# Autodesk Inventor assembly: Gearbox
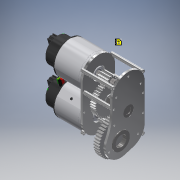
[picture p0: Inventor's stored thumbnail of the model, 180x180]
Saved by Autodesk Inventor 2019.4 (Build 234330000, 330)
## iProperties
Created: 2019-12-11
Part Number: Gearbox
Document SubType Name: Assembly
Designer: admin
Author: admin
## Documents named in this file (11)
- C:\Users\admin\Desktop\FRC 2020 Engineering\GitHub\Gearbox.iam
- C:\Users\admin\Desktop\FRC 2020 Engineering\GitHub\7738-CAD-prep\Swerve Module\Falcon_500_Powered_by_Talon_FX_217-6515.iam
- C:\Users\admin\Desktop\FRC 2020 Engineering\GitHub\7738-CAD-prep\WCD\10T_Steel_Spur_Gear_20_DP_12T_Center_Distance_Falcon_Motor_217-6917.ipt
- C:\Users\admin\Desktop\FRC 2020 Engineering\GitHub\40t_Aluminum_Spur_Gear_20_DP_1_2_Hex_Bore_217-2708.ipt
- C:\Users\admin\Desktop\FRC 2020 Engineering\GitHub\Gearbox\Design Accelerator\Spur Gears1.iam
- C:\Users\admin\Desktop\FRC 2020 Engineering\GitHub\7738-CAD-prep\Butterfly Drive Mk2\Butterfly Base\F6800Z 10mm ID Flange.ipt
- C:\Users\admin\Desktop\FRC 2020 Engineering\GitHub\Gearbox Plate 1.ipt
- C:\Users\admin\Desktop\FRC 2020 Engineering\GitHub\7738-CAD-prep\Butterfly Drive Mk2\Butterfly Module\F6004.ipt
- C:\Users\admin\Desktop\FRC 2020 Engineering\GitHub\Gearbox Plate 2.ipt
- C:\Users\admin\Desktop\FRC 2020 Engineering\GitHub\Shaft Jr.ipt
- C:\Users\admin\Desktop\FRC 2020 Engineering\GitHub\Spacer.ipt
## Components (18 placed, 10 different names)
1. Falcon_500_Powered_by_Talon_FX_217-6515:1 [sub-assembly] — Mate:2, Flush:1, Mate:5, Mate:7, Flush:4, Mate:11, Mate:15
2. Falcon_500_Powered_by_Talon_FX_217-6515:2 [sub-assembly] — Flush:1, Mate:3, Mate:4, Mate:6, Mate:9, Mate:13, Mate:14
3. 10T_Steel_Spur_Gear_20_DP_12T_Center_Distance_Falcon_Motor_217-6917:2 — Mate:2, Flush:2
4. 10T_Steel_Spur_Gear_20_DP_12T_Center_Distance_Falcon_Motor_217-6917:3 — Mate:3, Flush:2, Flush:3, Mate:9
5. 40t_Aluminum_Spur_Gear_20_DP_1_2_Hex_Bore_217-2708:1 — Flush:3, Mate:6, Mate:7, Mate:8, Mate:10
6. Spur Gears:1 [sub-assembly] — Mate:10, Mate:11, Mate:18, Mate:19, Mate:20
7. F6800Z 10mm ID Flange:1 — Mate:16, Mate:17, Mate:26
8. Gearbox Plate 1:1 — Mate:13, Mate:14, Mate:15, Mate:16, Mate:17
9. F6004:1 — Mate:21, Mate:22
10. Gearbox Plate 2:1 — Mate:19, Mate:20, Mate:21, Mate:22, Mate:23, Mate:24, Mate:27, Mate:28, Mate:29, Mate:30, Mate:31, Mate:32, Mate:33, Mate:34, Mate:35, Mate:36, Mate:37, Mate:38
11. F6800Z 10mm ID Flange:2 — Mate:23, Mate:24, Mate:25
12. Shaft Jr:1 — Mate:25, Mate:26
13. Spacer:1 — Mate:30, Mate:32
14. Spacer:2 — Mate:29, Mate:35
15. Spacer:3 — Mate:28, Mate:34
16. Spacer:4 — Mate:27, Mate:33
17. Spacer:5 — Mate:31, Mate:36
18. Spacer:6 — Mate:37, Mate:38
## Relationships (41: Mate 36, Flush 5)
- Mate:2: Falcon_500_Powered_by_Talon_FX_217-6515:1 ↔ 10T_Steel_Spur_Gear_20_DP_12T_Center_Distance_Falcon_Motor_217-6917:2
- Flush:1: Falcon_500_Powered_by_Talon_FX_217-6515:1 ↔ Falcon_500_Powered_by_Talon_FX_217-6515:2
- Mate:3: Falcon_500_Powered_by_Talon_FX_217-6515:2 ↔ 10T_Steel_Spur_Gear_20_DP_12T_Center_Distance_Falcon_Motor_217-6917:3
- Flush:2: 10T_Steel_Spur_Gear_20_DP_12T_Center_Distance_Falcon_Motor_217-6917:2 ↔ 10T_Steel_Spur_Gear_20_DP_12T_Center_Distance_Falcon_Motor_217-6917:3
- Mate:4: Falcon_500_Powered_by_Talon_FX_217-6515:2
- Mate:5: Falcon_500_Powered_by_Talon_FX_217-6515:1
- Flush:3 (5 mm): 10T_Steel_Spur_Gear_20_DP_12T_Center_Distance_Falcon_Motor_217-6917:3 ↔ 40t_Aluminum_Spur_Gear_20_DP_1_2_Hex_Bore_217-2708:1
- Mate:6 (33.02 mm): Falcon_500_Powered_by_Talon_FX_217-6515:2 ↔ 40t_Aluminum_Spur_Gear_20_DP_1_2_Hex_Bore_217-2708:1
- Mate:7 (33.02 mm): Falcon_500_Powered_by_Talon_FX_217-6515:1 ↔ 40t_Aluminum_Spur_Gear_20_DP_1_2_Hex_Bore_217-2708:1
- Flush:4: Falcon_500_Powered_by_Talon_FX_217-6515:1
- Mate:8: 40t_Aluminum_Spur_Gear_20_DP_1_2_Hex_Bore_217-2708:1
- Mate:9 (5 mm): Falcon_500_Powered_by_Talon_FX_217-6515:2 ↔ 10T_Steel_Spur_Gear_20_DP_12T_Center_Distance_Falcon_Motor_217-6917:3
- Mate:10: 40t_Aluminum_Spur_Gear_20_DP_1_2_Hex_Bore_217-2708:1 ↔ Spur Gears:1
- Mate:11 (5 mm): Falcon_500_Powered_by_Talon_FX_217-6515:1 ↔ Spur Gears:1
- Mate:13: Falcon_500_Powered_by_Talon_FX_217-6515:2 ↔ Gearbox Plate 1:1
- Mate:14: Falcon_500_Powered_by_Talon_FX_217-6515:2 ↔ Gearbox Plate 1:1
- Mate:15: Falcon_500_Powered_by_Talon_FX_217-6515:1 ↔ Gearbox Plate 1:1
- Mate:16 (0.2 mm): F6800Z 10mm ID Flange:1 ↔ Gearbox Plate 1:1
- Mate:17: F6800Z 10mm ID Flange:1 ↔ Gearbox Plate 1:1
- Flush:5 (-15 mm)
- Mate:18: Spur Gears:1
- Mate:19: Spur Gears:1 ↔ Gearbox Plate 2:1
- Mate:20 (5 mm): Spur Gears:1 ↔ Gearbox Plate 2:1
- Mate:21 (0.2 mm): F6004:1 ↔ Gearbox Plate 2:1
- Mate:22: F6004:1 ↔ Gearbox Plate 2:1
- Mate:23 (0.2 mm): Gearbox Plate 2:1 ↔ F6800Z 10mm ID Flange:2
- Mate:24: Gearbox Plate 2:1 ↔ F6800Z 10mm ID Flange:2
- Mate:25: F6800Z 10mm ID Flange:2 ↔ Shaft Jr:1
- Mate:26 (0.1 mm): F6800Z 10mm ID Flange:1 ↔ Shaft Jr:1
- Mate:27: Gearbox Plate 2:1 ↔ Spacer:4
- Mate:28: Gearbox Plate 2:1 ↔ Spacer:3
- Mate:29: Gearbox Plate 2:1 ↔ Spacer:2
- Mate:30: Gearbox Plate 2:1 ↔ Spacer:1
- Mate:31: Gearbox Plate 2:1 ↔ Spacer:5
- Mate:32 (0.1 mm): Gearbox Plate 2:1 ↔ Spacer:1
- Mate:33 (0.1 mm): Gearbox Plate 2:1 ↔ Spacer:4
- Mate:34 (0.1 mm): Gearbox Plate 2:1 ↔ Spacer:3
- Mate:35 (0.1 mm): Gearbox Plate 2:1 ↔ Spacer:2
- Mate:36 (0.1 mm): Gearbox Plate 2:1 ↔ Spacer:5
- Mate:37 (0.1 mm): Gearbox Plate 2:1 ↔ Spacer:6
- Mate:38: Gearbox Plate 2:1 ↔ Spacer:6
